# Autodesk Inventor assembly: power_train
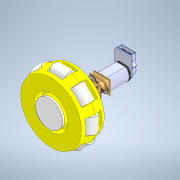
[picture p0: Inventor's stored thumbnail of the model, 180x180]
Saved by Autodesk Inventor 2020.4 (Build 244396000, 396)
## iProperties
Created: 2020-06-15
Part Number: power_train
Document SubType Name: Assembly
Designer: Tarsoly
Author: Tarsoly
## Documents named in this file (4)
- C:\Users\Tarsoly\Dokumentumok\BME\Dipterv\3d\power_train.iam
- C:\Users\Tarsoly\Dokumentumok\BME\Dipterv\3d\DC_GE_Motor\DC_GE_RED_Motor.iam
- C:\Users\Tarsoly\Dokumentumok\BME\Dipterv\3d\wheel_adapt.ipt
- C:\Users\Tarsoly\Dokumentumok\BME\Dipterv\3d\omniwheel_assembly.iam
## Components (3 placed, 3 different names)
1. DC_GE_RED_Motor:1 [sub-assembly] — Mate:5, Angle:2, Mate:6
2. wheel_adapt:1 — Mate:2, Angle:1, Mate:3, Mate:5, Mate:6
3. omniwheel_assembly:1 [sub-assembly] — Mate:1, Mate:2, Angle:1, Mate:3, Mate:4, Angle:3
## Relationships (9: Mate 6, Angle 3)
- Mate:1: omniwheel_assembly:1
- Mate:2: wheel_adapt:1 ↔ omniwheel_assembly:1
- Angle:1 (180 deg): wheel_adapt:1 ↔ omniwheel_assembly:1
- Mate:3: wheel_adapt:1 ↔ omniwheel_assembly:1
- Mate:4: omniwheel_assembly:1
- Mate:5: DC_GE_RED_Motor:1 ↔ wheel_adapt:1
- Angle:2 (0 deg): DC_GE_RED_Motor:1
- Mate:6 (3.7 mm): DC_GE_RED_Motor:1 ↔ wheel_adapt:1
- Angle:3 (180 deg): omniwheel_assembly:1
